# Autodesk Inventor assembly: tower_pro_mg-955
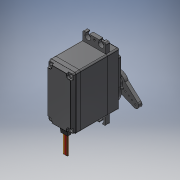
[picture p0: Inventor's stored thumbnail of the model, 180x180]
Saved by Autodesk Inventor 2017 (Build 210142000, 142)
## iProperties
Part Number: tower_pro_mg-955
Material: Ogólny
Document SubType Name: Assembly
Designer: Speed King
Author: Speed King
## Documents named in this file (3)
- C:\Users\Speed King\Documents\My Inventor\GrabCAD\Technical Informatics\CAD\model wstepny 17.04.26\Tower Pro MG955\tower_pro_mg-955.iam
- C:\Users\Speed King\Documents\My Inventor\GrabCAD\Technical Informatics\CAD\model wstepny 17.04.26\Tower Pro MG955\TOWER PRO MG-995, ANALOG SERVO.iam
- C:\Users\Speed King\Documents\My Inventor\GrabCAD\Technical Informatics\CAD\model wstepny 17.04.26\Tower Pro MG955\orczyk.ipt
## Components (2 placed, 2 different names)
1. TOWER PRO MG-995, ANALOG SERVO:1 [sub-assembly] — Zestawiający:1, Zestawiający:2
2. orczyk:1 — Zestawiający:1, Zestawiający:2
## Relationships (2: Mate 2)
- Zestawiający:1 [Mate]: TOWER PRO MG-995, ANALOG SERVO:1 ↔ orczyk:1
- Zestawiający:2 [Mate]: TOWER PRO MG-995, ANALOG SERVO:1 ↔ orczyk:1
